# Autodesk Inventor assembly: Assembly2
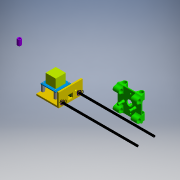
[picture p0: Inventor's stored thumbnail of the model, 180x180]
Saved by Autodesk Inventor 2016 (Build 200138000, 138)
## iProperties
Created: 2018-01-17
Part Number: Assembly2
Document SubType Name: Assembly
Designer: student
Author: student
## Documents named in this file (12)
- C:\gitHub_projects\Plotter_CAD\plotter_project\PLOTTER\Assembly2.iam
- C:\gitHub_projects\Plotter_CAD\plotter_project\PLOTTER\Part2.ipt
- C:\gitHub_projects\Plotter_CAD\plotter_project\PLOTTER\axis plotter motor timing pulley.ipt
- C:\gitHub_projects\Plotter_CAD\plotter_project\PLOTTER\Part3.ipt
- C:\gitHub_projects\Plotter_CAD\plotter_project\PLOTTER\Part9.ipt
- C:\gitHub_projects\Plotter_CAD\plotter_project\PLOTTER\Part14.ipt
- C:\gitHub_projects\Plotter_CAD\plotter_project\PLOTTER\Part15.ipt
- C:\gitHub_projects\Plotter_CAD\plotter_project\PLOTTER\Part16.ipt
- C:\gitHub_projects\Plotter_CAD\plotter_project\PLOTTER\Part10.ipt
- C:\gitHub_projects\Plotter_CAD\plotter_project\PLOTTER\rod.ipt
- C:\gitHub_projects\Plotter_CAD\plotter_project\PLOTTER\axis plotter berring mount.ipt
- C:\gitHub_projects\Plotter_CAD\plotter_project\PLOTTER\Part1.ipt
## Components (17 placed, 11 different names)
1. Part2:1 — Insert:1, Angle:3, Mate:1, Mate:2, Angle:5, Angle:10
2. axis plotter motor timing pulley:1 — Insert:1
3. Part3:1 — Mate:1, Mate:2, Rigid:1, Rigid:4, Angle:4, Flush:2, Rigid:5, Rigid:6
4. Part9:1 — Rigid:1
5. Part9:3 — Rigid:4
6. Part9:4 — Rigid:5
7. Part9:5 — Rigid:6, Flush:3
8. Part14:1 — Flush:3, Flush:4, Mate:5, Mate:8
9. Part15:1 — Flush:4, Mate:3, Mate:4, Mate:6, Mate:7, Rigid:9, Rigid:10
10. Part16:1 — Mate:3, Mate:4, Mate:5
11. Part16:2 — Mate:6, Mate:7, Mate:8
12. Part10:1 — Rigid:7, Rigid:10
13. rod:1 — Rigid:7
14. rod:2 — Rigid:8
15. Part10:2 — Rigid:8, Rigid:9
16. axis plotter berring mount:1
17. Part1:1
## Relationships (27: Mate 8, WeldJoint 8, Angle 6, Flush 4, Insert 1)
- Insert:1: Part2:1 ↔ axis plotter motor timing pulley:1
- Angle:3 (180 deg): Part2:1
- Mate:1: Part2:1 ↔ Part3:1
- Mate:2: Part2:1 ↔ Part3:1
- Rigid:1 [WeldJoint]: Part3:1 ↔ Part9:1
- Rigid:4 [WeldJoint]: Part3:1 ↔ Part9:3
- Angle:4 (0 deg): Part3:1
- Flush:1 (-56 mm)
- Angle:5 (0 deg): Part2:1
- Flush:2 (30 mm): Part3:1
- Angle:8 (0 deg)
- Angle:9 (0 deg)
- Rigid:5 [WeldJoint]: Part3:1 ↔ Part9:4
- Rigid:6 [WeldJoint]: Part3:1 ↔ Part9:5
- Flush:3: Part9:5 ↔ Part14:1
- Flush:4: Part14:1 ↔ Part15:1
- Angle:10 (0 deg): Part2:1
- Mate:3: Part15:1 ↔ Part16:1
- Mate:4: Part15:1 ↔ Part16:1
- Mate:5: Part14:1 ↔ Part16:1
- Mate:6: Part15:1 ↔ Part16:2
- Mate:7: Part15:1 ↔ Part16:2
- Mate:8: Part14:1 ↔ Part16:2
- Rigid:7 [WeldJoint]: Part10:1 ↔ rod:1
- Rigid:8 [WeldJoint]: rod:2 ↔ Part10:2
- Rigid:9 [WeldJoint]: Part15:1 ↔ Part10:2
- Rigid:10 [WeldJoint]: Part15:1 ↔ Part10:1
